# Autodesk Inventor assembly: Összeállítás
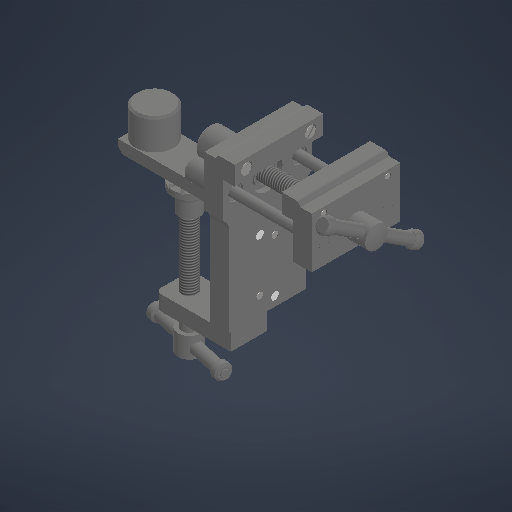
[picture p0: Inventor's stored thumbnail of the model, 512x512]
Saved by Autodesk Inventor 2025 (Build 290162010, 162A)
## iProperties
Created: 2025-02-13
Part Number: Összeállítás
Document SubType Name: Assembly
Designer: petruska.milan
Author: petruska.milan
## Documents named in this file (20)
- C:\Users\petruska.milan\Documents\pmproject\Összeállítás.iam
- C:\Users\petruska.milan\Documents\pmproject\Gyűrű.ipt
- C:\Users\petruska.milan\Documents\pmproject\Hajtókar1.ipt
- C:\Users\petruska.milan\Documents\pmproject\Hajtókar2.ipt
- C:\Users\petruska.milan\Documents\pmproject\Kengyel2.ipt
- C:\Users\petruska.milan\Documents\pmproject\Meneteshüvely.ipt
- C:\Users\petruska.milan\Documents\pmproject\Menetesorsó.ipt
- C:\Users\petruska.milan\Documents\pmproject\Mozgatóorsó.ipt
- C:\Users\petruska.milan\Documents\pmproject\Nyomódarab.ipt
- C:\Users\petruska.milan\Documents\pmproject\Satupofa.ipt
- C:\Users\petruska.milan\Documents\pmproject\Szorítólap.ipt
- C:\Users\petruska.milan\Documents\pmproject\üllő.ipt
- C:\Users\petruska.milan\Documents\pmproject\Vezetőhüvely.ipt
- C:\Users\petruska.milan\Documents\pmproject\Kengyel3.ipt
- C:\Users\petruska.milan\Documents\pmproject\Lap2.ipt
- C:\Users\petruska.milan\Documents\pmproject\vezetőcsap.ipt
- C:\Users\petruska.milan\Documents\pmproject\illesztőszög.ipt
- C:\Users\petruska.milan\Documents\pmproject\illesztőcsap.ipt
- C:\Users\petruska.milan\Documents\Inventor\Content Center Files\R2025\en-US\ISO 1207(2)\ISO 1207 - M4 x 14.ipt
- C:\Users\petruska.milan\Documents\Inventor\Content Center Files\R2025\en-US\ISO 1207(2)\ISO 1207 - M3 x 14.ipt
## Components (28 placed, 19 different names)
1. Gyűrű:1 — Mate:4, Mate:5
2. Hajtókar1:1 — Mate:27, Mate:28, Mate:29, Tangent:2
3. Hajtókar2:1 — Mate:3, Mate:4, Mate:5, Mate:33
4. Kengyel2:1 — Flush:1, Mate:1, Flush:2, Mate:2, Mate:34
5. Kengyel3:1 — Flush:1, Mate:1, Flush:2, Mate:6, Mate:7, Mate:8, Mate:9, Mate:10, Mate:36, Mate:37, Mate:38, Mate:39
6. Lap2:1 — Mate:8, Mate:9, Mate:10, Mate:11, Mate:12, Mate:13, Mate:14, Mate:22, Mate:23, Mate:24, Mate:25, Mate:26, Flush:5, Flush:6, Flush:7, Flush:8, Mate:42, Mate:43, Flush:10, Flush:11
7. Meneteshüvely:1 — Mate:21, Mate:22
8. Menetesorsó:1 — Mate:2, Mate:3, Mate:20, Tangent:1, Mate:33, Mate:34
9. Mozgatóorsó:1 — Mate:11, Mate:15, Mate:16, Mate:21, Mate:27, Tangent:2
10. Nyomódarab:1 — Mate:20, Tangent:1, Mate:32, Tangent:3
11. Szorítólap:1 — Mate:15, Angle:1, Mate:16, Mate:17, Mate:18, Mate:19, Mate:30, Mate:31, Flush:3, Flush:4, Flush:9, Flush:12
12. üllő:1 — Mate:6, Mate:7
13. Vezetőhüvely:1 — Mate:23, Mate:25
14. Satupofa:1 — Mate:12, Mate:13, Mate:14, Angle:1, Mate:35
15. Satupofa:2 — Mate:17, Mate:18, Mate:19, Mate:35, Mate:40, Mate:41
16. Vezetőhüvely:2 — Mate:24, Mate:26
17. Gyűrű:2 — Mate:28, Mate:29
18. vezetőcsap:1 — Mate:31, Flush:4
19. vezetőcsap:2 — Mate:30, Flush:3
20. illesztőszög:1 — Mate:32, Tangent:3
21. illesztőcsap:1 — Mate:36, Flush:6
22. illesztőcsap:2 — Mate:37, Flush:5
23. ISO 1207 M4 x 14:1 — Mate:39, Flush:7
24. ISO 1207 M4 x 14:2 — Mate:38, Flush:8
25. ISO 1207 M3 x 14:1 — Mate:41, Flush:12
26. ISO 1207 M3 x 14:2 — Mate:43, Flush:10
27. ISO 1207 M3 x 14:3 — Mate:40, Flush:9
28. ISO 1207 M3 x 14:4 — Mate:42, Flush:11
## Relationships (59: Mate 43, Flush 12, Tangent 3, Angle 1)
- Flush:1: Kengyel2:1 ↔ Kengyel3:1
- Mate:1: Kengyel2:1 ↔ Kengyel3:1
- Flush:2: Kengyel2:1 ↔ Kengyel3:1
- Mate:2: Kengyel2:1 ↔ Menetesorsó:1
- Mate:3: Hajtókar2:1 ↔ Menetesorsó:1
- Mate:4: Gyűrű:1 ↔ Hajtókar2:1
- Mate:5: Gyűrű:1 ↔ Hajtókar2:1
- Mate:6: Kengyel3:1 ↔ üllő:1
- Mate:7: Kengyel3:1 ↔ üllő:1
- Mate:8: Kengyel3:1 ↔ Lap2:1
- Mate:9: Kengyel3:1 ↔ Lap2:1
- Mate:10: Kengyel3:1 ↔ Lap2:1
- Mate:11: Lap2:1 ↔ Mozgatóorsó:1
- Mate:12: Lap2:1 ↔ Satupofa:1
- Mate:13: Lap2:1 ↔ Satupofa:1
- Mate:14: Lap2:1 ↔ Satupofa:1
- Mate:15: Mozgatóorsó:1 ↔ Szorítólap:1
- Angle:1 (0 deg): Szorítólap:1 ↔ Satupofa:1
- Mate:16: Mozgatóorsó:1 ↔ Szorítólap:1
- Mate:17: Szorítólap:1 ↔ Satupofa:2
- Mate:18: Szorítólap:1 ↔ Satupofa:2
- Mate:19: Szorítólap:1 ↔ Satupofa:2
- Mate:20: Menetesorsó:1 ↔ Nyomódarab:1
- Tangent:1: Menetesorsó:1 ↔ Nyomódarab:1
- Mate:21: Meneteshüvely:1 ↔ Mozgatóorsó:1
- Mate:22: Lap2:1 ↔ Meneteshüvely:1
- Mate:23: Lap2:1 ↔ Vezetőhüvely:1
- Mate:24: Lap2:1 ↔ Vezetőhüvely:2
- Mate:25: Lap2:1 ↔ Vezetőhüvely:1
- Mate:26: Lap2:1 ↔ Vezetőhüvely:2
- Mate:27: Hajtókar1:1 ↔ Mozgatóorsó:1
- Mate:28: Hajtókar1:1 ↔ Gyűrű:2
- Mate:29: Hajtókar1:1 ↔ Gyűrű:2
- Mate:30: Szorítólap:1 ↔ vezetőcsap:2
- Mate:31: Szorítólap:1 ↔ vezetőcsap:1
- Flush:3: Szorítólap:1 ↔ vezetőcsap:2
- Flush:4: Szorítólap:1 ↔ vezetőcsap:1
- Mate:32: Nyomódarab:1 ↔ illesztőszög:1
- Mate:33 (25 mm): Hajtókar2:1 ↔ Menetesorsó:1
- Mate:34 (9 mm): Kengyel2:1 ↔ Menetesorsó:1
- Mate:35: Satupofa:1 ↔ Satupofa:2
- Tangent:2 (23 mm): Hajtókar1:1 ↔ Mozgatóorsó:1
- Mate:36: Kengyel3:1 ↔ illesztőcsap:1
- Mate:37: Kengyel3:1 ↔ illesztőcsap:2
- Flush:5: Lap2:1 ↔ illesztőcsap:2
- Flush:6: Lap2:1 ↔ illesztőcsap:1
- Mate:38: Kengyel3:1 ↔ ISO 1207 M4 x 14:2
- Mate:39: Kengyel3:1 ↔ ISO 1207 M4 x 14:1
- Flush:7: Lap2:1 ↔ ISO 1207 M4 x 14:1
- Flush:8: Lap2:1 ↔ ISO 1207 M4 x 14:2
- Mate:40: Satupofa:2 ↔ ISO 1207 M3 x 14:3
- Flush:9: Szorítólap:1 ↔ ISO 1207 M3 x 14:3
- Mate:41: Satupofa:2 ↔ ISO 1207 M3 x 14:1
- Mate:42: Lap2:1 ↔ ISO 1207 M3 x 14:4
- Mate:43: Lap2:1 ↔ ISO 1207 M3 x 14:2
- Flush:10: Lap2:1 ↔ ISO 1207 M3 x 14:2
- Flush:11: Lap2:1 ↔ ISO 1207 M3 x 14:4
- Flush:12: Szorítólap:1 ↔ ISO 1207 M3 x 14:1
- Tangent:3 (-9.5 mm): Nyomódarab:1 ↔ illesztőszög:1
